# Autodesk Inventor assembly: NXT assembly
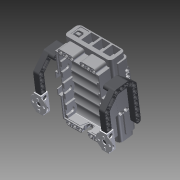
[picture p0: Inventor's stored thumbnail of the model, 180x180]
Saved by Autodesk Inventor 2014 SP2 (Build 180246200, 246)
## iProperties
Created: 2014-11-05
Part Number: NXT assembly
Document SubType Name: Assembly
Designer: Allison
Author: Allison
## Documents named in this file (4)
- C:\Users\Allison\Documents\inventor\InventorMasterProject\NXT assembly.iam
- C:\Users\Allison\Documents\inventor\InventorMasterProject\Lego\CPU and battery\NXT Body.ipt
- C:\Users\Allison\Documents\inventor\InventorMasterProject\Lego\Beams\beam_angle_9x5.ipt
- C:\Users\Allison\Documents\inventor\InventorMasterProject\Tetrix\Lego hardpoint mount\Lego Mounting Hub.ipt
## Components (7 placed, 3 different names)
1. NXT Body:1 — Insert:4, Insert:5, Insert:8, Flush:3
2. beam_angle_9x5:1 — Insert:1, Flush:1, Insert:3, Mate:1
3. beam_angle_9x5:2 — Insert:1, Flush:1, Insert:4, Insert:5
4. beam_angle_9x5:4 — Insert:6, Mate:2, Insert:7, Flush:2
5. Lego Mounting Hub:1 — Insert:3, Mate:1
6. Lego Mounting Hub:2 — Insert:6, Mate:2
7. beam_angle_9x5:5 — Insert:7, Flush:2, Insert:8, Flush:3
## Relationships (12: Insert 7, Flush 3, Mate 2)
- Insert:1: beam_angle_9x5:1 ↔ beam_angle_9x5:2
- Flush:1: beam_angle_9x5:1 ↔ beam_angle_9x5:2
- Insert:3: beam_angle_9x5:1 ↔ Lego Mounting Hub:1
- Mate:1: beam_angle_9x5:1 ↔ Lego Mounting Hub:1
- Insert:4: NXT Body:1 ↔ beam_angle_9x5:2
- Insert:5: NXT Body:1 ↔ beam_angle_9x5:2
- Insert:6: beam_angle_9x5:4 ↔ Lego Mounting Hub:2
- Mate:2: beam_angle_9x5:4 ↔ Lego Mounting Hub:2
- Insert:7: beam_angle_9x5:4 ↔ beam_angle_9x5:5
- Flush:2: beam_angle_9x5:4 ↔ beam_angle_9x5:5
- Insert:8: NXT Body:1 ↔ beam_angle_9x5:5
- Flush:3: NXT Body:1 ↔ beam_angle_9x5:5
